# Autodesk Inventor assembly: Conmcept 4-Assembly
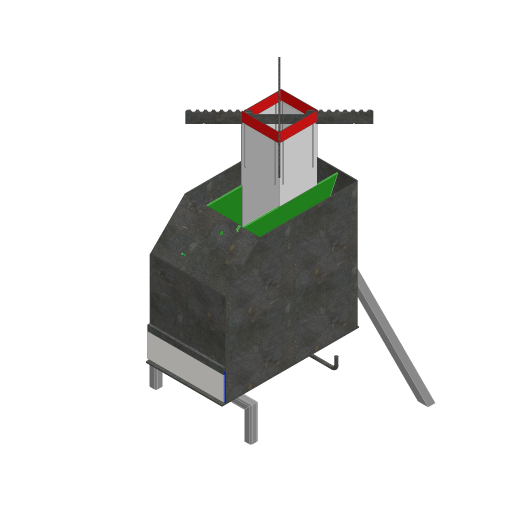
[picture p0: Inventor's stored thumbnail of the model, 512x512]
Saved by Autodesk Inventor 2024.3 (Build 283343000, 343)
## iProperties
Created: 2025-06-17
Part Number: Conmcept 4-Assembly
Document SubType Name: Assembly
Designer: ajclo
Mass: 21970.2 g
Surface Area: 16652 cm^2
Volume: 1937.41 cm^3
Density: 11.34 g/cm^3
Author: ajclo
## Documents named in this file (23)
- C:\Users\ajclo\OneDrive - Stellenbosch University\Documents\BEng\Year IV\Skripsie\CAD\CAD Final Design\Conmcept 4-Assembly.iam
- C:\Users\ajclo\OneDrive - Stellenbosch University\Documents\BEng\Year IV\Skripsie\CAD\CAD Final Design\FLU-ShaftRS3.ipt
- C:\Users\ajclo\OneDrive - Stellenbosch University\Documents\BEng\Year IV\Skripsie\CAD\CAD Final Design\LzC-FrontPLateRS3.ipt
- C:\Users\ajclo\OneDrive - Stellenbosch University\Documents\BEng\Year IV\Skripsie\CAD\CAD Final Design\LzC-StoveCover.ipt
- C:\Users\ajclo\OneDrive - Stellenbosch University\Documents\BEng\Year IV\Skripsie\CAD\CAD Final Design\WI-ShaftRS3.ipt
- C:\Users\ajclo\OneDrive - Stellenbosch University\Documents\BEng\Year IV\Skripsie\CAD\CAD Final Design\BottomPlateRS3.ipt
- C:\Users\ajclo\OneDrive - Stellenbosch University\Documents\BEng\Year IV\Skripsie\CAD\CAD Final Design\AI-RS3.ipt
- C:\Users\ajclo\OneDrive - Stellenbosch University\Documents\BEng\Year IV\Skripsie\CAD\CAD Final Design\FootRS3.iam
- C:\Users\ajclo\OneDrive - Stellenbosch University\Documents\BEng\Year IV\Skripsie\CAD\CAD Final Design\Flu-Expansion-RS3.ipt
- C:\Users\ajclo\OneDrive - Stellenbosch University\Documents\BEng\Year IV\Skripsie\CAD\CAD Final Design\Flu-ExpansionSidesRS3.ipt
- C:\Users\ajclo\OneDrive - Stellenbosch University\Documents\BEng\Year IV\Skripsie\CAD\CAD Final Design\Grid RS3.ipt
- C:\Users\ajclo\OneDrive - Stellenbosch University\Documents\BEng\Year IV\Skripsie\CAD\CAD Final Design\CapRS3.ipt
- C:\Users\ajclo\OneDrive - Stellenbosch University\Documents\BEng\Year IV\Skripsie\CAD\CAD Final Design\RS3_TubeFoot.ipt
- C:\Users\ajclo\OneDrive - Stellenbosch University\Documents\BEng\Year IV\Skripsie\CAD\CAD Final Design\pin.ipt
- C:\Users\ajclo\OneDrive - Stellenbosch University\Documents\BEng\Year IV\Skripsie\CAD\CAD Final Design\WI-Cover.ipt
- C:\Users\ajclo\OneDrive - Stellenbosch University\Documents\BEng\Year IV\Skripsie\CAD\CAD Final Design\AI-Cover.ipt
- C:\Users\ajclo\OneDrive - Stellenbosch University\Documents\BEng\Year IV\Skripsie\CAD\CAD Final Design\StoveTopAssembly.ipt.iam
- C:\Users\ajclo\OneDrive - Stellenbosch University\Documents\BEng\Year IV\Skripsie\CAD\CAD Final Design\GuiderailRS3.ipt
- C:\Users\ajclo\OneDrive - Stellenbosch University\Documents\BEng\Year IV\Skripsie\CAD\CAD Final Design\GuiderodsRS3.ipt
- C:\Users\ajclo\OneDrive - Stellenbosch University\Documents\BEng\Year IV\Skripsie\CAD\CAD Final Design\AllenKey-RS3.ipt
- C:\Users\ajclo\OneDrive - Stellenbosch University\Documents\BEng\Year IV\Skripsie\CAD\CAD Final Design\FLueExtension.ipt
- C:\Users\ajclo\OneDrive - Stellenbosch University\Documents\BEng\Year IV\Skripsie\CAD\CAD Final Design\ConstructionPlane1.ipt
- StoveTopAssembly.ipt
## Components (27 placed, 21 different names)
1. FLU-ShaftRS3:1 — Mate:1, Flush:1, Mate:5, Mate:6, Mate:7, Mate:10, Mate:17, Flush:7, Angle:1, Mate:19, Mate:21, Mate:68, Mate:69, Mate:70, Mate:71, Mate:76, Mate:77, Mate:80
2. LzC-FrontPLateRS3:1 — Flush:2, Mate:3, Mate:4, Mate:16, Mate:42, Mate:43, Mate:62, Mate:65
3. LzC-StoveCover:1 — Mate:8, Flush:3, Flush:4, Mate:11, Mate:29, Mate:30, Flush:25
4. WI-ShaftRS3:1 — Mate:1, Flush:1, Flush:2, Mate:3, Mate:4, Mate:31, Mate:39, Flush:21
5. BottomPlateRS3:1 — Mate:5, Mate:6, Mate:7, Mate:8, Flush:3, Flush:4, Mate:9, Mate:15, Mate:66, Mate:67, Flush:28
6. AI-RS3:1 — Mate:9, Mate:10, Mate:11
7. FootRS3:1 [sub-assembly] — Mate:15, Mate:16, Flush:15
8. Flu-Expansion-RS3:1 — Mate:17, Flush:7, Angle:1, Mate:18, Mate:20, Flush:9, Flush:10
9. Flu-ExpansionSidesRS3:1 — Mate:18, Mate:19, Flush:10, Mate:31, Mate:79
10. Flu-ExpansionSidesRS3:2 — Mate:20, Mate:21, Flush:9
11. Grid RS3:1 — Flush:28, Mate:76, Mate:77
12. RS3_TubeFoot:1 — Flush:14, Mate:29, Mate:78
13. RS3_TubeFoot:2 — Flush:14, Flush:15, Mate:30, Mate:78
14. pin:1 — Mate:39, Flush:21, Mate:41, Mate:43
15. WI-Cover:1 — Mate:41, Mate:42
16. CapRS3:1 — Mate:68, Mate:69, Mate:73, Mate:74, Mate:75
17. AI-Cover:1 — Mate:62, Mate:67
18. StoveTopAssembly.ipt:1 [sub-assembly] — Mate:81, Mate:82, Mate:83
19. GuiderailRS3:1 — Flush:25, Mate:65, Mate:66
20. GuiderodsRS3:1 — Flush:26, Flush:27, Mate:71, Mate:72
21. GuiderodsRS3:2 — Flush:26, Mate:70, Flush:27, Mate:72
22. AllenKey-RS3:1 — Mate:73, Mate:74, Mate:75
23. FLueExtension:1 — Mate:79, Mate:80, Mate:81, Mate:82, Mate:83, Mate:86, Mate:87, Mate:88, Mate:89
24. ConstructionPlane1:1 — Flush:29, Mate:86
25. ConstructionPlane1:2 — Flush:29, Flush:30, Mate:87
26. ConstructionPlane1:3 — Flush:30, Flush:31, Mate:88
27. ConstructionPlane1:4 — Flush:31, Mate:89
## Relationships (66: Mate 48, Flush 17, Angle 1)
- Mate:1: FLU-ShaftRS3:1 ↔ WI-ShaftRS3:1
- Flush:1: FLU-ShaftRS3:1 ↔ WI-ShaftRS3:1
- Flush:2: LzC-FrontPLateRS3:1 ↔ WI-ShaftRS3:1
- Mate:3: LzC-FrontPLateRS3:1 ↔ WI-ShaftRS3:1
- Mate:4: LzC-FrontPLateRS3:1 ↔ WI-ShaftRS3:1
- Mate:5: FLU-ShaftRS3:1 ↔ BottomPlateRS3:1
- Mate:6: FLU-ShaftRS3:1 ↔ BottomPlateRS3:1
- Mate:7: FLU-ShaftRS3:1 ↔ BottomPlateRS3:1
- Mate:8: LzC-StoveCover:1 ↔ BottomPlateRS3:1
- Flush:3: LzC-StoveCover:1 ↔ BottomPlateRS3:1
- Flush:4: LzC-StoveCover:1 ↔ BottomPlateRS3:1
- Mate:9: BottomPlateRS3:1 ↔ AI-RS3:1
- Mate:10: FLU-ShaftRS3:1 ↔ AI-RS3:1
- Mate:11: LzC-StoveCover:1 ↔ AI-RS3:1
- Mate:15: BottomPlateRS3:1 ↔ FootRS3:1
- Mate:16 (-50 mm): LzC-FrontPLateRS3:1 ↔ FootRS3:1
- Mate:17: FLU-ShaftRS3:1 ↔ Flu-Expansion-RS3:1
- Flush:7: FLU-ShaftRS3:1 ↔ Flu-Expansion-RS3:1
- Angle:1 (25 deg): FLU-ShaftRS3:1 ↔ Flu-Expansion-RS3:1
- Mate:18: Flu-Expansion-RS3:1 ↔ Flu-ExpansionSidesRS3:1
- Mate:19: FLU-ShaftRS3:1 ↔ Flu-ExpansionSidesRS3:1
- Mate:20: Flu-Expansion-RS3:1 ↔ Flu-ExpansionSidesRS3:2
- Mate:21: FLU-ShaftRS3:1 ↔ Flu-ExpansionSidesRS3:2
- Flush:9: Flu-Expansion-RS3:1 ↔ Flu-ExpansionSidesRS3:2
- Flush:10: Flu-Expansion-RS3:1 ↔ Flu-ExpansionSidesRS3:1
- Flush:14: RS3_TubeFoot:1 ↔ RS3_TubeFoot:2
- Mate:29: LzC-StoveCover:1 ↔ RS3_TubeFoot:1
- Flush:15: FootRS3:1 ↔ RS3_TubeFoot:2
- Mate:30 (-100 mm): LzC-StoveCover:1 ↔ RS3_TubeFoot:2
- Mate:31: WI-ShaftRS3:1 ↔ Flu-ExpansionSidesRS3:1
- Mate:39: WI-ShaftRS3:1 ↔ pin:1
- Flush:21: WI-ShaftRS3:1 ↔ pin:1
- Mate:41: pin:1 ↔ WI-Cover:1
- Mate:42 (1 mm): LzC-FrontPLateRS3:1 ↔ WI-Cover:1
- Mate:43 (73.6 mm): LzC-FrontPLateRS3:1 ↔ pin:1
- Mate:62: LzC-FrontPLateRS3:1 ↔ AI-Cover:1
- Flush:25: LzC-StoveCover:1 ↔ GuiderailRS3:1
- Mate:65: LzC-FrontPLateRS3:1 ↔ GuiderailRS3:1
- Mate:66 (80 mm): BottomPlateRS3:1 ↔ GuiderailRS3:1
- Mate:67: BottomPlateRS3:1 ↔ AI-Cover:1
- Mate:68: FLU-ShaftRS3:1 ↔ CapRS3:1
- Mate:69: FLU-ShaftRS3:1 ↔ CapRS3:1
- Flush:26: GuiderodsRS3:1 ↔ GuiderodsRS3:2
- Mate:70 (-13 mm): FLU-ShaftRS3:1 ↔ GuiderodsRS3:2
- Flush:27: GuiderodsRS3:1 ↔ GuiderodsRS3:2
- Mate:71: FLU-ShaftRS3:1 ↔ GuiderodsRS3:1
- Mate:72 (50 mm): GuiderodsRS3:1 ↔ GuiderodsRS3:2
- Mate:73: CapRS3:1 ↔ AllenKey-RS3:1
- Mate:74: CapRS3:1 ↔ AllenKey-RS3:1
- Mate:75 (44.5 mm): CapRS3:1 ↔ AllenKey-RS3:1
- Flush:28: BottomPlateRS3:1 ↔ Grid RS3:1
- Mate:76: FLU-ShaftRS3:1 ↔ Grid RS3:1
- Mate:77: FLU-ShaftRS3:1 ↔ Grid RS3:1
- Mate:78: RS3_TubeFoot:1 ↔ RS3_TubeFoot:2
- Mate:79: Flu-ExpansionSidesRS3:1 ↔ FLueExtension:1
- Mate:80: FLU-ShaftRS3:1 ↔ FLueExtension:1
- Mate:81: StoveTopAssembly.ipt:1 ↔ FLueExtension:1
- Mate:82: StoveTopAssembly.ipt:1 ↔ FLueExtension:1
- Mate:83: StoveTopAssembly.ipt:1 ↔ FLueExtension:1
- Flush:29: ConstructionPlane1:1 ↔ ConstructionPlane1:2
- Flush:30: ConstructionPlane1:2 ↔ ConstructionPlane1:3
- Flush:31: ConstructionPlane1:3 ↔ ConstructionPlane1:4
- Mate:86: FLueExtension:1 ↔ ConstructionPlane1:1
- Mate:87: FLueExtension:1 ↔ ConstructionPlane1:2
- Mate:88: FLueExtension:1 ↔ ConstructionPlane1:3
- Mate:89: FLueExtension:1 ↔ ConstructionPlane1:4
